# Autodesk Inventor assembly: pryBar
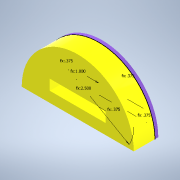
[picture p0: Inventor's stored thumbnail of the model, 180x180]
Saved by Autodesk Inventor 2021.1 (Build 251245000, 245)
## iProperties
Created: 2020-09-14
Part Number: pryBar
Document SubType Name: Assembly
Designer: robst
Author: robst
## Documents named in this file (3)
- C:\git\CAD-Development\robSteele\ShapeWays\ToolBelt\pryBar.iam
- C:\git\CAD-Development\robSteele\ShapeWays\ToolBelt\dRingHolder.ipt
- C:\git\CAD-Development\robSteele\ShapeWays\ToolBelt\dRingHolderBottom.ipt
## Components (2 placed, 2 different names)
1. dRingHolder:1 — Mate:1, Mate:2
2. dRingHolderBottom:1 — Mate:1, Mate:2
## Relationships (2: Mate 2)
- Mate:1: dRingHolder:1 ↔ dRingHolderBottom:1
- Mate:2: dRingHolder:1 ↔ dRingHolderBottom:1
